# Autodesk Inventor assembly: Intake
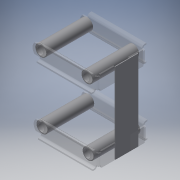
[picture p0: Inventor's stored thumbnail of the model, 180x180]
Saved by Autodesk Inventor 2018 (Build 220112000, 112)
## iProperties
Created: 2018-01-16
Part Number: Intake
Document SubType Name: Assembly
Designer: brooksprench
Author: brooksprench
## Documents named in this file (3)
- C:\Users\uzair\Documents\School\Clubs\Robotics\CAD for Unity\Intake.iam
- C:\Users\uzair\Documents\School\Clubs\Robotics\2018Robot\4992 Robot v0.2\4992-2018-Intake - Single Side.iam
- C:\Users\uzair\Documents\School\Clubs\Robotics\2018Robot\4992 Robot v0.2\4992-2018-Intake Mount Plate.ipt
## Components (3 placed, 2 different names)
1. 4992-2018-Intake - Single Side:1 [sub-assembly] — Flush:1, Flush:2
2. 4992-2018-Intake - Single Side:2 [sub-assembly] — Flush:3, Mate:1, Mate:2
3. 4992-2018-Intake Mount Plate:1 — Flush:1, Flush:2, Flush:3, Mate:1, Mate:2
## Relationships (5: Flush 3, Mate 2)
- Flush:1: 4992-2018-Intake - Single Side:1 ↔ 4992-2018-Intake Mount Plate:1
- Flush:2: 4992-2018-Intake - Single Side:1 ↔ 4992-2018-Intake Mount Plate:1
- Flush:3: 4992-2018-Intake - Single Side:2 ↔ 4992-2018-Intake Mount Plate:1
- Mate:1: 4992-2018-Intake - Single Side:2 ↔ 4992-2018-Intake Mount Plate:1
- Mate:2: 4992-2018-Intake - Single Side:2 ↔ 4992-2018-Intake Mount Plate:1
